# Autodesk Inventor assembly: 計測輪周り
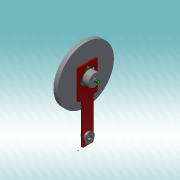
[picture p0: Inventor's stored thumbnail of the model, 180x180]
Saved by Autodesk Inventor 2015 (Build 190159000, 159)
## iProperties
Created: 2016-04-05
Part Number: 計測輪周り
Document SubType Name: Assembly
Designer: buzztaka
Author: buzztaka
## Documents named in this file (16)
- C:\Users\buzztaka\Downloads\2kk\計測輪周り.iam
- C:\Users\buzztaka\Downloads\2kk\kw\C-SFL6901ZZ.ipt
- C:\Users\buzztaka\Downloads\2kk\kw\meh-30-pエンコーダ.ipt
- C:\Users\buzztaka\Downloads\2kk\kw\スプリングフランジ用ワッシャー（座金）.ipt
- C:\Users\buzztaka\Downloads\2kk\kw\スプリングフランジ0.1mm.ipt
- C:\Users\buzztaka\Downloads\2kk\CapboltM5-8.ipt
- C:\Users\buzztaka\Downloads\2kk\washer M5.ipt
- C:\Users\buzztaka\Downloads\2kk\WSSS16-12-(ワッシャ12mm).ipt
- C:\Users\buzztaka\Downloads\2kk\低頭ネジｍ3 6mm\CBSH3-6.ipt
- C:\Users\buzztaka\Downloads\2kk\kw\タイヤアーム.ipt
- C:\Users\buzztaka\Downloads\2kk\m3ワッシャ\PACK-PWFN3.ipt
- C:\Users\buzztaka\Downloads\2kk\m3　10mm　低頭\CBS3-10.ipt
- C:\Users\buzztaka\Downloads\2kk\m3ナット\SLBNR3.ipt
- C:\Users\buzztaka\Downloads\2kk\計測輪20mm.ipt
- C:\Users\buzztaka\Downloads\2kk\12mmホルダフランジ改\SSTHRT12-MB_b.ipt
- C:\Users\buzztaka\Downloads\2kk\回転アーム付き計測輪シャフト - コピー.ipt
## Components (29 placed, 15 different names)
1. C-SFL6901ZZ:2 — 挿入:17, 挿入:32
2. meh-30-pエンコーダ:1 — 挿入:42
3. スプリングフランジ用ワッシャー（座金）:1
4. スプリングフランジ用ワッシャー（座金）:2
5. スプリングフランジ用ワッシャー（座金）:3 — 挿入:23
6. スプリングフランジ0.1mm:1 — 挿入:21, 挿入:22, 挿入:30, 挿入:31, 挿入:36, 挿入:37, 挿入:38
7. CapboltM5-8:1 — 挿入:44
8. washer M5:1 — 挿入:43, 挿入:44
9. WSSS16-12-(ワッシャ12mm):1 — 挿入:17, 挿入:39
10. CBSH3-6:1 — 挿入:23
11. CBSH3-6:2 — 挿入:22
12. CBSH3-6:3 — 挿入:21
13. タイヤアーム:1 — 挿入:24, 挿入:25, 挿入:26, 挿入:32, 挿入:33, 挿入:34, 挿入:35, 挿入:40
14. PACK-PWFN3:1 — 挿入:24, 挿入:27
15. PACK-PWFN3:6 — 挿入:29, 挿入:31
16. PACK-PWFN3:7 — 挿入:26, 挿入:29
17. PACK-PWFN3:8 — 挿入:27, 挿入:30
18. PACK-PWFN3:9 — 挿入:28
19. PACK-PWFN3:10 — 挿入:25, 挿入:28
20. CBS3-10:1 — 挿入:33
21. CBS3-10:2 — 挿入:34
22. CBS3-10:3 — 挿入:35
23. SLBNR3:1 — 挿入:37
24. SLBNR3:2 — 挿入:38
25. SLBNR3:3 — 挿入:36
26. 計測輪20mm:1 — 挿入:39
27. WSSS16-12-(ワッシャ12mm):2 — 挿入:41
28. SSTHRT12-MB_b:1 — 挿入:40, 挿入:41
29. 回転アーム付き計測輪シャフト - コピー:1 — 挿入:42, 挿入:43
## Relationships (30: Insert 30)
- [Insert]: meh-30-pエンコーダ:1 ↔ スプリングフランジ用ワッシャー（座金）:2
- [Insert]: meh-30-pエンコーダ:1 ↔ スプリングフランジ用ワッシャー（座金）:1
- [Insert]: meh-30-pエンコーダ:1 ↔ スプリングフランジ用ワッシャー（座金）:3
- [Insert]: スプリングフランジ用ワッシャー（座金）:2 ↔ スプリングフランジ0.1mm:1
- [Insert]: スプリングフランジ用ワッシャー（座金）:3 ↔ スプリングフランジ0.1mm:1
- 挿入:17 [Insert]: C-SFL6901ZZ:2 ↔ WSSS16-12-(ワッシャ12mm):1
- 挿入:21 [Insert]: スプリングフランジ0.1mm:1 ↔ CBSH3-6:3
- 挿入:22 [Insert]: スプリングフランジ0.1mm:1 ↔ CBSH3-6:2
- 挿入:23 [Insert]: スプリングフランジ用ワッシャー（座金）:3 ↔ CBSH3-6:1
- 挿入:24 [Insert]: タイヤアーム:1 ↔ PACK-PWFN3:1
- 挿入:25 [Insert]: タイヤアーム:1 ↔ PACK-PWFN3:10
- 挿入:26 [Insert]: タイヤアーム:1 ↔ PACK-PWFN3:7
- 挿入:27 [Insert]: PACK-PWFN3:1 ↔ PACK-PWFN3:8
- 挿入:28 [Insert]: PACK-PWFN3:9 ↔ PACK-PWFN3:10
- 挿入:29 [Insert]: PACK-PWFN3:6 ↔ PACK-PWFN3:7
- 挿入:30 [Insert]: スプリングフランジ0.1mm:1 ↔ PACK-PWFN3:8
- 挿入:31 [Insert]: スプリングフランジ0.1mm:1 ↔ PACK-PWFN3:6
- 挿入:32 [Insert]: C-SFL6901ZZ:2 ↔ タイヤアーム:1
- 挿入:33 [Insert]: タイヤアーム:1 ↔ CBS3-10:1
- 挿入:34 [Insert]: タイヤアーム:1 ↔ CBS3-10:2
- 挿入:35 [Insert]: タイヤアーム:1 ↔ CBS3-10:3
- 挿入:36 [Insert]: スプリングフランジ0.1mm:1 ↔ SLBNR3:3
- 挿入:37 [Insert]: スプリングフランジ0.1mm:1 ↔ SLBNR3:1
- 挿入:38 [Insert]: スプリングフランジ0.1mm:1 ↔ SLBNR3:2
- 挿入:39 [Insert]: WSSS16-12-(ワッシャ12mm):1 ↔ 計測輪20mm:1
- 挿入:40 [Insert]: タイヤアーム:1 ↔ SSTHRT12-MB_b:1
- 挿入:41 [Insert]: WSSS16-12-(ワッシャ12mm):2 ↔ SSTHRT12-MB_b:1
- 挿入:42 [Insert] (-10 mm): meh-30-pエンコーダ:1 ↔ 回転アーム付き計測輪シャフト - コピー:1
- 挿入:43 [Insert]: washer M5:1 ↔ 回転アーム付き計測輪シャフト - コピー:1
- 挿入:44 [Insert]: CapboltM5-8:1 ↔ washer M5:1
